# Autodesk Inventor assembly: Assembly_Omniscope_v1
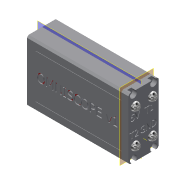
[picture p0: Inventor's stored thumbnail of the model, 180x180]
Saved by Autodesk Inventor 2019 (Build 230136000, 136)
## iProperties
Created: 2021-09-22
Part Number: Assembly_Omniscope_v1
Material: Generisch
Document SubType Name: Assembly
Designer: Muriel
Mass: 21.4058 g
Surface Area: 211.771 cm^2
Volume: 21.4058 cm^3
Density: 1 g/cm^3
Author: Muriel
## Documents named in this file (7)
- C:\Users\Muriel\Documents\Inventor\HITscope\Assembly_Omniscope_v1.iam
- C:\Users\Muriel\Documents\Inventor\HITscope\01_Camera_Module_left_v0.ipt
- C:\Users\Muriel\Documents\Inventor\HITscope\01_Camera_Module_Lit.ipt
- C:\Users\Muriel\Documents\Inventor\HITscope\00_ESP32_Board.ipt
- C:\Users\Muriel\Documents\Inventor\HITscope\03_Camera_Clip.ipt
- C:\Users\Muriel\Documents\Inventor\HITscope\02_Camera_Lid.ipt
- C:\Users\Muriel\Documents\Inventor\HITscope\00_Ballmagnet_5mm.ipt
## Components (10 placed, 6 different names)
1. 01_Camera_Module_left_v0:1 — Fluchtend:2, Einfügen:2, Fluchtend:3, Einfügen:3, Fluchtend:4, Fluchtend:5
2. 01_Camera_Module_Lit:1 — Fluchtend:2
3. 00_ESP32_Board:1 — Einfügen:2
4. 00_ESP32_Board:2 — Einfügen:3
5. 03_Camera_Clip:1 — Fluchtend:3
6. 02_Camera_Lid:1 — Fluchtend:4, Fluchtend:5, Passend:1, Passend:2, Passend:3, Passend:4
7. 00_Ballmagnet_5mm:1 — Passend:4
8. 00_Ballmagnet_5mm:2 — Passend:2
9. 00_Ballmagnet_5mm:3 — Passend:1
10. 00_Ballmagnet_5mm:4 — Passend:3
## Relationships (10: Flush 4, Mate 4, Insert 2)
- Fluchtend:2 [Flush]: 01_Camera_Module_left_v0:1 ↔ 01_Camera_Module_Lit:1
- Einfügen:2 [Insert]: 01_Camera_Module_left_v0:1 ↔ 00_ESP32_Board:1
- Fluchtend:3 [Flush]: 01_Camera_Module_left_v0:1 ↔ 03_Camera_Clip:1
- Einfügen:3 [Insert]: 01_Camera_Module_left_v0:1 ↔ 00_ESP32_Board:2
- Fluchtend:4 [Flush]: 01_Camera_Module_left_v0:1 ↔ 02_Camera_Lid:1
- Fluchtend:5 [Flush]: 01_Camera_Module_left_v0:1 ↔ 02_Camera_Lid:1
- Passend:1 [Mate]: 02_Camera_Lid:1 ↔ 00_Ballmagnet_5mm:3
- Passend:2 [Mate]: 02_Camera_Lid:1 ↔ 00_Ballmagnet_5mm:2
- Passend:3 [Mate]: 02_Camera_Lid:1 ↔ 00_Ballmagnet_5mm:4
- Passend:4 [Mate]: 02_Camera_Lid:1 ↔ 00_Ballmagnet_5mm:1
